# Autodesk Inventor assembly: bottle jigsaw assembly
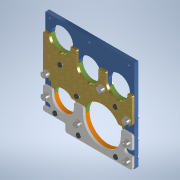
[picture p0: Inventor's stored thumbnail of the model, 180x180]
Saved by Autodesk Inventor 2021 (Build 250183000, 183)
## iProperties
Created: 2020-08-07
Part Number: bottle jigsaw assembly
Document SubType Name: Assembly
Designer: jgray
Author: jgray
## Documents named in this file (12)
- M:\Printed Electronics\Gas Sensors\Prototypes\Prototype II -Cartridge Reader V3\bottle jigsaw assembly.iam
- M:\Printed Electronics\Gas Sensors\Prototypes\Prototype II -Cartridge Reader V3\Bottle clamping plate 1.ipt
- M:\Printed Electronics\Gas Sensors\Prototypes\Prototype II -Cartridge Reader V3\Bottle clamping plate 2.ipt
- M:\Printed Electronics\Gas Sensors\Prototypes\Prototype II -Cartridge Reader V3\Bottle layout.ipt
- M:\Printed Electronics\Gas Sensors\Prototypes\Prototype II -Cartridge Reader V3\Bottle layout pt3.ipt
- M:\Printed Electronics\Gas Sensors\Prototypes\Prototype II -Cartridge Reader V3\Bottle layout pt2.ipt
- C:\Users\jgray\Documents\Inventor\Content Center Files\R2021\en-US\ISO 4762(2)\ISO 4762 - M4 x 12ISO.ipt
- C:\Users\jgray\Documents\Inventor\Content Center Files\R2021\en-US\DIN 6798  J\DIN 6798 - J 4.3.ipt
- C:\Users\jgray\Documents\Inventor\Content Center Files\R2021\en-US\DIN 934\DIN 934 - M4 x 0.7.ipt
- M:\Printed Electronics\Gas Sensors\Prototypes\Prototype II -Cartridge Reader V3\RS 278-534 M3 fixing Dia4FixHole.ipt
- C:\Users\jgray\Documents\Inventor\Content Center Files\R2021\en-US\ISO 7380-1\ISO 7380-1 - M3 x 10.ipt
- C:\Users\jgray\Documents\Inventor\Content Center Files\R2021\en-US\DIN 6798  J\DIN 6798 - J 3.2.ipt
## Components (51 placed, 11 different names)
1. Bottle clamping plate 1:1 — Mate:5, Mate:6, Mate:23, Mate:25, Mate:28, Mate:29, Mate:30, Mate:31, Mate:35, Mate:37, Mate:79, Mate:80, Mate:81, Mate:85, Mate:86, Mate:87, Mate:94
2. Bottle clamping plate 2:1 — Mate:3, Mate:4, Mate:22, Mate:26, Mate:27, Mate:33, Mate:34, Mate:76, Mate:77, Mate:78, Mate:82, Mate:83, Mate:84, Flush:8
3. Bottle layout:1 — Flush:1, Mate:1, Mate:8, Mate:9, Mate:10, Mate:11, Mate:12, Mate:13, Mate:15, Mate:16, Mate:18, Mate:19, Mate:20, Mate:32, Mate:102, Mate:103, Flush:8, Mate:106, Angle:1
4. Bottle layout pt3:1 — Mate:2, Mate:5, Mate:6, Flush:2, Mate:70, Mate:74, Mate:75, Flush:3, Flush:6, Mate:101, Mate:104, Mate:105, Flush:9
5. Bottle layout pt2:1 — Flush:1, Mate:1, Mate:2, Mate:3, Mate:4, Mate:14, Mate:71, Mate:72, Mate:73, Flush:4, Flush:5, Flush:7, Mate:102, Mate:103, Mate:104, Mate:105, Flush:9
6. ISO 4762 M4 x 12:2 — Mate:42, Mate:49, Mate:65, Mate:108
7. ISO 4762 M4 x 12:3 — Mate:39, Mate:51, Mate:67
8. ISO 4762 M4 x 12:4 — Mate:38, Mate:50, Mate:66
9. ISO 4762 M4 x 12:5 — Mate:45, Mate:46, Mate:62
10. ISO 4762 M4 x 12:6 — Mate:44, Mate:47, Mate:63
11. ISO 4762 M4 x 12:7 — Mate:43, Mate:48, Mate:64
12. ISO 4762 M4 x 12:8 — Mate:41, Mate:53, Mate:68, Mate:107
13. DIN 6798 J J 4.3:1 — Mate:27, Mate:32, Mate:43, Mate:48
14. DIN 6798 J J 4.3:2 — Mate:28, Mate:31, Mate:44, Mate:47
15. DIN 6798 J J 4.3:3 — Mate:14, Mate:57, Mate:107
16. DIN 6798 J J 4.3:4 — Mate:26, Mate:33, Mate:42, Mate:49
17. DIN 6798 J J 4.3:5 — Mate:29, Mate:30, Mate:45, Mate:46
18. DIN 6798 J J 4.3:6 — Mate:9, Mate:15, Mate:56
19. DIN 6798 J J 4.3:7 — Mate:12, Mate:18, Mate:59
20. DIN 6798 J J 4.3:8 — Mate:13, Mate:58, Mate:108
21. DIN 6798 J J 4.3:9 — Mate:10, Mate:20, Mate:61
22. DIN 6798 J J 4.3:10 — Mate:11, Mate:19, Mate:60
23. DIN 6798 J J 4.3:11 — Mate:8, Mate:16, Mate:55
24. DIN 934 - replaced by DIN EN 24032/28673/28674 M4:2 — Mate:59, Mate:64
25. DIN 934 - replaced by DIN EN 24032/28673/28674 M4:3 — Mate:57, Mate:68
26. DIN 934 - replaced by DIN EN 24032/28673/28674 M4:4 — Mate:56, Mate:66
27. DIN 934 - replaced by DIN EN 24032/28673/28674 M4:5 — Mate:55, Mate:67
28. DIN 934 - replaced by DIN EN 24032/28673/28674 M4:7 — Mate:61, Mate:62
29. DIN 934 - replaced by DIN EN 24032/28673/28674 M4:8 — Mate:60, Mate:63
30. DIN 934 - replaced by DIN EN 24032/28673/28674 M4:9 — Mate:58, Mate:65
31. DIN 6798 J J 4.3:13 — Mate:25, Mate:37, Mate:41, Mate:53
32. DIN 6798 J J 4.3:14 — Mate:23, Mate:35, Mate:39, Mate:51
33. DIN 6798 J J 4.3:15 — Mate:22, Mate:34, Mate:38, Mate:50
34. RS 278-534 M3 fixing Dia4FixHole:3 — Flush:2, Mate:70, Mate:100
35. RS 278-534 M3 fixing Dia4FixHole:10 — Mate:71, Flush:7
36. RS 278-534 M3 fixing Dia4FixHole:11 — Mate:73, Flush:5
37. RS 278-534 M3 fixing Dia4FixHole:12 — Mate:74, Flush:6
38. RS 278-534 M3 fixing Dia4FixHole:13 — Mate:75, Flush:3
39. RS 278-534 M3 fixing Dia4FixHole:14 — Mate:72, Flush:4
40. ISO 7380-1 M3 x 10:1 — Mate:90, Mate:95
41. ISO 7380-1 M3 x 10:2 — Mate:93, Mate:94, Mate:101
42. ISO 7380-1 M3 x 10:3 — Mate:89, Mate:96, Mate:100
43. ISO 7380-1 M3 x 10:4 — Mate:92, Mate:99
44. ISO 7380-1 M3 x 10:5 — Mate:88, Mate:97
45. ISO 7380-1 M3 x 10:6 — Mate:91, Mate:98
46. DIN 6798 J J 3.2:1 — Mate:76, Mate:83, Mate:92, Mate:99
47. DIN 6798 J J 3.2:2 — Mate:81, Mate:86, Mate:90, Mate:95
48. DIN 6798 J J 3.2:3 — Mate:78, Mate:84, Mate:88, Mate:97
49. DIN 6798 J J 3.2:4 — Mate:77, Mate:82, Mate:91, Mate:98
50. DIN 6798 J J 3.2:5 — Mate:80, Mate:85, Mate:89, Mate:96
51. DIN 6798 J J 3.2:6 — Mate:79, Mate:87, Mate:93
## Relationships (109: Mate 99, Flush 9, Angle 1)
- Flush:1: Bottle layout:1 ↔ Bottle layout pt2:1
- Mate:1: Bottle layout:1 ↔ Bottle layout pt2:1
- Mate:2: Bottle layout pt3:1 ↔ Bottle layout pt2:1
- Mate:3: Bottle clamping plate 2:1 ↔ Bottle layout pt2:1
- Mate:4: Bottle clamping plate 2:1 ↔ Bottle layout pt2:1
- Mate:5: Bottle clamping plate 1:1 ↔ Bottle layout pt3:1
- Mate:6: Bottle clamping plate 1:1 ↔ Bottle layout pt3:1
- Mate:8: Bottle layout:1 ↔ DIN 6798 J J 4.3:11
- Mate:9: Bottle layout:1 ↔ DIN 6798 J J 4.3:6
- Mate:10: Bottle layout:1 ↔ DIN 6798 J J 4.3:9
- Mate:11: Bottle layout:1 ↔ DIN 6798 J J 4.3:10
- Mate:12: Bottle layout:1 ↔ DIN 6798 J J 4.3:7
- Mate:13: Bottle layout:1 ↔ DIN 6798 J J 4.3:8
- Mate:14: Bottle layout pt2:1 ↔ DIN 6798 J J 4.3:3
- Mate:15: Bottle layout:1 ↔ DIN 6798 J J 4.3:6
- Mate:16: Bottle layout:1 ↔ DIN 6798 J J 4.3:11
- Mate:18: Bottle layout:1 ↔ DIN 6798 J J 4.3:7
- Mate:19: Bottle layout:1 ↔ DIN 6798 J J 4.3:10
- Mate:20: Bottle layout:1 ↔ DIN 6798 J J 4.3:9
- Mate:22: Bottle clamping plate 2:1 ↔ DIN 6798 J J 4.3:15
- Mate:23: Bottle clamping plate 1:1 ↔ DIN 6798 J J 4.3:14
- Mate:25: Bottle clamping plate 1:1 ↔ DIN 6798 J J 4.3:13
- Mate:26: Bottle clamping plate 2:1 ↔ DIN 6798 J J 4.3:4
- Mate:27: Bottle clamping plate 2:1 ↔ DIN 6798 J J 4.3:1
- Mate:28: Bottle clamping plate 1:1 ↔ DIN 6798 J J 4.3:2
- Mate:29: Bottle clamping plate 1:1 ↔ DIN 6798 J J 4.3:5
- Mate:30: Bottle clamping plate 1:1 ↔ DIN 6798 J J 4.3:5
- Mate:31: Bottle clamping plate 1:1 ↔ DIN 6798 J J 4.3:2
- Mate:32: Bottle layout:1 ↔ DIN 6798 J J 4.3:1
- Mate:33: Bottle clamping plate 2:1 ↔ DIN 6798 J J 4.3:4
- Mate:34: Bottle clamping plate 2:1 ↔ DIN 6798 J J 4.3:15
- Mate:35: Bottle clamping plate 1:1 ↔ DIN 6798 J J 4.3:14
- Mate:37: Bottle clamping plate 1:1 ↔ DIN 6798 J J 4.3:13
- Mate:38: ISO 4762 M4 x 12:4 ↔ DIN 6798 J J 4.3:15
- Mate:39: ISO 4762 M4 x 12:3 ↔ DIN 6798 J J 4.3:14
- Mate:41: ISO 4762 M4 x 12:8 ↔ DIN 6798 J J 4.3:13
- Mate:42: ISO 4762 M4 x 12:2 ↔ DIN 6798 J J 4.3:4
- Mate:43: ISO 4762 M4 x 12:7 ↔ DIN 6798 J J 4.3:1
- Mate:44: ISO 4762 M4 x 12:6 ↔ DIN 6798 J J 4.3:2
- Mate:45: ISO 4762 M4 x 12:5 ↔ DIN 6798 J J 4.3:5
- Mate:46: ISO 4762 M4 x 12:5 ↔ DIN 6798 J J 4.3:5
- Mate:47: ISO 4762 M4 x 12:6 ↔ DIN 6798 J J 4.3:2
- Mate:48: ISO 4762 M4 x 12:7 ↔ DIN 6798 J J 4.3:1
- Mate:49: ISO 4762 M4 x 12:2 ↔ DIN 6798 J J 4.3:4
- Mate:50: ISO 4762 M4 x 12:4 ↔ DIN 6798 J J 4.3:15
- Mate:51: ISO 4762 M4 x 12:3 ↔ DIN 6798 J J 4.3:14
- Mate:53: ISO 4762 M4 x 12:8 ↔ DIN 6798 J J 4.3:13
- Mate:55: DIN 6798 J J 4.3:11 ↔ DIN 934 - replaced by DIN EN 24032/28673/28674 M4:5
- Mate:56: DIN 6798 J J 4.3:6 ↔ DIN 934 - replaced by DIN EN 24032/28673/28674 M4:4
- Mate:57: DIN 6798 J J 4.3:3 ↔ DIN 934 - replaced by DIN EN 24032/28673/28674 M4:3
- Mate:58: DIN 6798 J J 4.3:8 ↔ DIN 934 - replaced by DIN EN 24032/28673/28674 M4:9
- Mate:59: DIN 6798 J J 4.3:7 ↔ DIN 934 - replaced by DIN EN 24032/28673/28674 M4:2
- Mate:60: DIN 6798 J J 4.3:10 ↔ DIN 934 - replaced by DIN EN 24032/28673/28674 M4:8
- Mate:61: DIN 6798 J J 4.3:9 ↔ DIN 934 - replaced by DIN EN 24032/28673/28674 M4:7
- Mate:62: ISO 4762 M4 x 12:5 ↔ DIN 934 - replaced by DIN EN 24032/28673/28674 M4:7
- Mate:63: ISO 4762 M4 x 12:6 ↔ DIN 934 - replaced by DIN EN 24032/28673/28674 M4:8
- Mate:64: ISO 4762 M4 x 12:7 ↔ DIN 934 - replaced by DIN EN 24032/28673/28674 M4:2
- Mate:65: ISO 4762 M4 x 12:2 ↔ DIN 934 - replaced by DIN EN 24032/28673/28674 M4:9
- Mate:66: ISO 4762 M4 x 12:4 ↔ DIN 934 - replaced by DIN EN 24032/28673/28674 M4:4
- Mate:67: ISO 4762 M4 x 12:3 ↔ DIN 934 - replaced by DIN EN 24032/28673/28674 M4:5
- Mate:68: ISO 4762 M4 x 12:8 ↔ DIN 934 - replaced by DIN EN 24032/28673/28674 M4:3
- Flush:2: Bottle layout pt3:1 ↔ RS 278-534 M3 fixing Dia4FixHole:3
- Mate:70: Bottle layout pt3:1 ↔ RS 278-534 M3 fixing Dia4FixHole:3
- Mate:71: Bottle layout pt2:1 ↔ RS 278-534 M3 fixing Dia4FixHole:10
- Mate:72: Bottle layout pt2:1 ↔ RS 278-534 M3 fixing Dia4FixHole:14
- Mate:73: Bottle layout pt2:1 ↔ RS 278-534 M3 fixing Dia4FixHole:11
- Mate:74: Bottle layout pt3:1 ↔ RS 278-534 M3 fixing Dia4FixHole:12
- Mate:75: Bottle layout pt3:1 ↔ RS 278-534 M3 fixing Dia4FixHole:13
- Flush:3: Bottle layout pt3:1 ↔ RS 278-534 M3 fixing Dia4FixHole:13
- Flush:4: Bottle layout pt2:1 ↔ RS 278-534 M3 fixing Dia4FixHole:14
- Flush:5: Bottle layout pt2:1 ↔ RS 278-534 M3 fixing Dia4FixHole:11
- Flush:6: Bottle layout pt3:1 ↔ RS 278-534 M3 fixing Dia4FixHole:12
- Flush:7: Bottle layout pt2:1 ↔ RS 278-534 M3 fixing Dia4FixHole:10
- Mate:76: Bottle clamping plate 2:1 ↔ DIN 6798 J J 3.2:1
- Mate:77: Bottle clamping plate 2:1 ↔ DIN 6798 J J 3.2:4
- Mate:78: Bottle clamping plate 2:1 ↔ DIN 6798 J J 3.2:3
- Mate:79: Bottle clamping plate 1:1 ↔ DIN 6798 J J 3.2:6
- Mate:80: Bottle clamping plate 1:1 ↔ DIN 6798 J J 3.2:5
- Mate:81: Bottle clamping plate 1:1 ↔ DIN 6798 J J 3.2:2
- Mate:82: Bottle clamping plate 2:1 ↔ DIN 6798 J J 3.2:4
- Mate:83: Bottle clamping plate 2:1 ↔ DIN 6798 J J 3.2:1
- Mate:84: Bottle clamping plate 2:1 ↔ DIN 6798 J J 3.2:3
- Mate:85: Bottle clamping plate 1:1 ↔ DIN 6798 J J 3.2:5
- Mate:86: Bottle clamping plate 1:1 ↔ DIN 6798 J J 3.2:2
- Mate:87: Bottle clamping plate 1:1 ↔ DIN 6798 J J 3.2:6
- Mate:88: ISO 7380-1 M3 x 10:5 ↔ DIN 6798 J J 3.2:3
- Mate:89: ISO 7380-1 M3 x 10:3 ↔ DIN 6798 J J 3.2:5
- Mate:90: ISO 7380-1 M3 x 10:1 ↔ DIN 6798 J J 3.2:2
- Mate:91: ISO 7380-1 M3 x 10:6 ↔ DIN 6798 J J 3.2:4
- Mate:92: ISO 7380-1 M3 x 10:4 ↔ DIN 6798 J J 3.2:1
- Mate:93: ISO 7380-1 M3 x 10:2 ↔ DIN 6798 J J 3.2:6
- Mate:94: Bottle clamping plate 1:1 ↔ ISO 7380-1 M3 x 10:2
- Mate:95: ISO 7380-1 M3 x 10:1 ↔ DIN 6798 J J 3.2:2
- Mate:96: ISO 7380-1 M3 x 10:3 ↔ DIN 6798 J J 3.2:5
- Mate:97: ISO 7380-1 M3 x 10:5 ↔ DIN 6798 J J 3.2:3
- Mate:98: ISO 7380-1 M3 x 10:6 ↔ DIN 6798 J J 3.2:4
- Mate:99: ISO 7380-1 M3 x 10:4 ↔ DIN 6798 J J 3.2:1
- Mate:100: RS 278-534 M3 fixing Dia4FixHole:3 ↔ ISO 7380-1 M3 x 10:3
- Mate:101: Bottle layout pt3:1 ↔ ISO 7380-1 M3 x 10:2
- Mate:102: Bottle layout:1 ↔ Bottle layout pt2:1
- Mate:103: Bottle layout:1 ↔ Bottle layout pt2:1
- Mate:104: Bottle layout pt3:1 ↔ Bottle layout pt2:1
- Mate:105: Bottle layout pt3:1 ↔ Bottle layout pt2:1
- Flush:8: Bottle clamping plate 2:1 ↔ Bottle layout:1
- Mate:106: Bottle layout:1
- Angle:1 (0 deg): Bottle layout:1
- Flush:9: Bottle layout pt3:1 ↔ Bottle layout pt2:1
- Mate:107: ISO 4762 M4 x 12:8 ↔ DIN 6798 J J 4.3:3
- Mate:108: ISO 4762 M4 x 12:2 ↔ DIN 6798 J J 4.3:8
